# Autodesk Inventor assembly: hingedPair
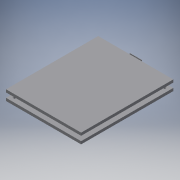
[picture p0: Inventor's stored thumbnail of the model, 180x180]
Saved by Autodesk Inventor 2019 (Build 230136000, 136)
## iProperties
Created: 2018-10-04
Part Number: hingedPair
Document SubType Name: Assembly
Designer: abhay
Author: abhay
## Documents named in this file (3)
- C:\Users\abhay\Documents\AuxArrayCAD\hingedPair.iam
- C:\Users\abhay\Documents\AuxArrayCAD\WoodFrame.ipt
- C:\Users\abhay\Documents\AuxArrayCAD\Hinge.ipt
## Components (3 placed, 2 different names)
1. WoodFrame:1 — Insert:1, Insert:2, Angle:1
2. Hinge:1 — Insert:1, Insert:2, Angle:1, Insert:3, Insert:4
3. WoodFrame:2 — Insert:3, Insert:4
## Relationships (5: Insert 4, Angle 1)
- Insert:1: WoodFrame:1 ↔ Hinge:1
- Insert:2: WoodFrame:1 ↔ Hinge:1
- Angle:1 (0 deg): WoodFrame:1 ↔ Hinge:1
- Insert:3: Hinge:1 ↔ WoodFrame:2
- Insert:4: Hinge:1 ↔ WoodFrame:2
